# Autodesk Inventor assembly: Calorimeter
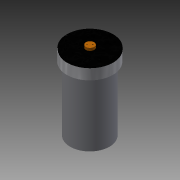
[picture p0: Inventor's stored thumbnail of the model, 180x180]
Saved by Autodesk Inventor 2014 (Build 180170000, 170)
## iProperties
Created: 2014-06-11
Part Number: Calorimeter
Document SubType Name: Assembly
Designer: Nabeel
Author: Nabeel
## Documents named in this file (5)
- C:\Users\Nabeel\Desktop\Nabu Stuff\VERL Work\Calorimeter\Calorimeter.iam
- C:\Users\Nabeel\Desktop\Nabu Stuff\VERL Work\Calorimeter\Outter Cup.ipt
- C:\Users\Nabeel\Desktop\Nabu Stuff\VERL Work\Calorimeter\Inner Cup.ipt
- C:\Users\Nabeel\Desktop\Nabu Stuff\VERL Work\Calorimeter\Plastic Lid.ipt
- C:\Users\Nabeel\Desktop\Nabu Stuff\VERL Work\Calorimeter\Rubber Stopper.ipt
## Components (4 placed, 4 different names)
1. Outter Cup:1 — Mate:1, Mate:3
2. Inner Cup:1 — Mate:1, Mate:2
3. Plastic Lid:1 — Mate:2, Mate:3, Insert:1
4. Rubber Stopper:1 — Insert:1
## Relationships (4: Mate 3, Insert 1)
- Mate:1: Outter Cup:1 ↔ Inner Cup:1
- Mate:2: Inner Cup:1 ↔ Plastic Lid:1
- Mate:3: Outter Cup:1 ↔ Plastic Lid:1
- Insert:1: Plastic Lid:1 ↔ Rubber Stopper:1
